# Autodesk Inventor assembly: Arm
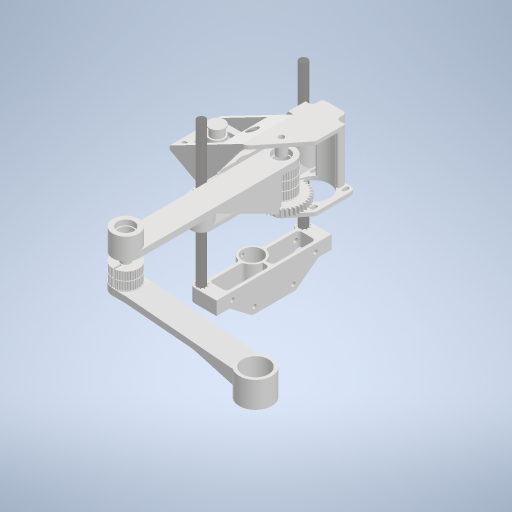
[picture p0: Inventor's stored thumbnail of the model, 512x512]
Saved by Autodesk Inventor 2024 (Build 280153000, 153)
## iProperties
Created: 2024-03-27
Part Number: Arm
Document SubType Name: Assembly
Designer: drew
Author: drew
## Documents named in this file (10)
- C:\Users\drew\Sync\CSCE 462\Arm.iam
- C:\Users\drew\Sync\CSCE 462\Arm Base stand.ipt
- C:\Users\drew\Sync\CSCE 462\Shaft.ipt
- C:\Users\drew\Sync\CSCE 462\gantry.ipt
- C:\Users\drew\Sync\CSCE 462\small pulley.ipt
- C:\Users\drew\Sync\CSCE 462\40t pulley.ipt
- C:\Users\drew\Sync\CSCE 462\inner arm.ipt
- C:\Users\drew\Sync\CSCE 462\top spacer.ipt
- C:\Users\drew\Sync\CSCE 462\bottom spacer.ipt
- C:\Users\drew\Sync\CSCE 462\outer arm.ipt
## Components (10 placed, 9 different names)
1. Arm Base stand:1 — Flush:1, Flush:2, Insert:1, Flush:3, Insert:2
2. Shaft:1 — Flush:2, Insert:2
3. Shaft:2 — Insert:1
4. gantry:1 — Flush:4, Flush:5, Mate:1, Flush:8
5. small pulley:1 — Flush:5, Flush:6
6. 40t pulley:1 — Flush:6, Mate:1, Insert:3
7. inner arm:1 — Insert:3, Flush:7, Insert:4
8. top spacer:1 — Flush:7
9. bottom spacer:1 — Flush:8
10. outer arm:1 — Insert:4
## Relationships (13: Flush 8, Insert 4, Mate 1)
- Flush:1: Arm Base stand:1
- Flush:2: Arm Base stand:1 ↔ Shaft:1
- Insert:1: Arm Base stand:1 ↔ Shaft:2
- Flush:3 (50.8 mm): Arm Base stand:1
- Flush:4: gantry:1
- Insert:2: Arm Base stand:1 ↔ Shaft:1
- Flush:5: gantry:1 ↔ small pulley:1
- Flush:6: small pulley:1 ↔ 40t pulley:1
- Mate:1: gantry:1 ↔ 40t pulley:1
- Insert:3: 40t pulley:1 ↔ inner arm:1
- Flush:7: inner arm:1 ↔ top spacer:1
- Flush:8: gantry:1 ↔ bottom spacer:1
- Insert:4: inner arm:1 ↔ outer arm:1
